# Autodesk Inventor assembly: P1704_E003_button
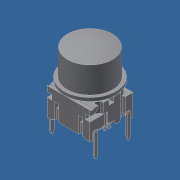
[picture p0: Inventor's stored thumbnail of the model, 180x180]
Saved by Autodesk Inventor 2019 (Build 230136000, 136)
## iProperties
Created: 2019-06-03
Part Number: P1704_E003_button
Project: Nom Projet
Description: Ens. Nom Ensemble
Document SubType Name: Assembly
Designer: Adel.KAHRIMANOVIC
Author: Adel.KAHRIMANOVIC
## Documents named in this file (3)
- P:\projet_manette\manette\06_Dessins\2019\Manette universelle\P1704_E003_button.iam
- P:\projet_manette\manette\06_Dessins\2019\Manette universelle\P1704_016_Button.ipt
- P:\projet_manette\manette\06_Dessins\2019\Manette universelle\P1704_017_button_cap.ipt
## Components (2 placed, 2 different names)
1. P1704_016_Button:1 — Placage:1, Placage:2
2. P1704_017_button_cap:1 — Placage:1, Placage:2
## Relationships (2: Mate 2)
- Placage:1 [Mate]: P1704_016_Button:1 ↔ P1704_017_button_cap:1
- Placage:2 [Mate]: P1704_016_Button:1 ↔ P1704_017_button_cap:1
